# Autodesk Inventor assembly: Full Tentacle
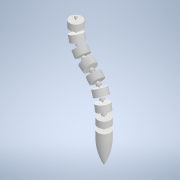
[picture p0: Inventor's stored thumbnail of the model, 180x180]
Saved by Autodesk Inventor 2021 (Build 250183000, 183)
## iProperties
Created: 2020-07-11
Part Number: Full Tentacle
Document SubType Name: Assembly
Designer: saipr
Author: saipr
## Documents named in this file (3)
- C:\Users\saipr\Desktop\Autodesk 2021\Builds\Parts\Full Tentacle.iam
- C:\Users\saipr\Desktop\Autodesk 2021\Builds\Parts\octopus tentacles.ipt
- C:\Users\saipr\Desktop\Autodesk 2021\Builds\Parts\octopus tentacle end.ipt
## Components (9 placed, 2 different names)
1. octopus tentacles:1 — Mate:1
2. octopus tentacles:2 — Mate:1, Mate:2
3. octopus tentacles:3 — Mate:2, Mate:3
4. octopus tentacles:4 — Mate:3, Mate:4
5. octopus tentacles:5 — Mate:4, Mate:5
6. octopus tentacles:6 — Mate:5, Mate:6
7. octopus tentacles:7 — Mate:6, Mate:7
8. octopus tentacles:8 — Mate:7, Mate:8
9. octopus tentacle end:1 — Mate:8
## Relationships (8: Mate 8)
- Mate:1: octopus tentacles:1 ↔ octopus tentacles:2
- Mate:2: octopus tentacles:2 ↔ octopus tentacles:3
- Mate:3: octopus tentacles:3 ↔ octopus tentacles:4
- Mate:4: octopus tentacles:4 ↔ octopus tentacles:5
- Mate:5: octopus tentacles:5 ↔ octopus tentacles:6
- Mate:6: octopus tentacles:6 ↔ octopus tentacles:7
- Mate:7: octopus tentacles:7 ↔ octopus tentacles:8
- Mate:8: octopus tentacles:8 ↔ octopus tentacle end:1
